# Autodesk Inventor assembly: ASY TZS 1200 Filter column D1200
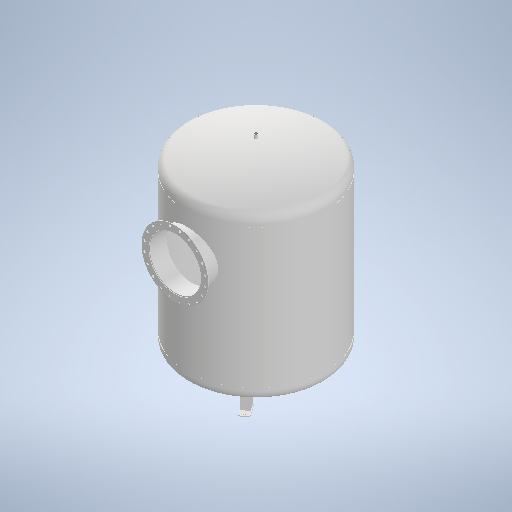
[picture p0: Inventor's stored thumbnail of the model, 512x512]
Saved by Autodesk Inventor 2025 (Build 290162010, 162A)
## iProperties
Created: 2025-02-13
Part Number: ASY TZS 1200 Filter column D1200
Document SubType Name: Assembly
Designer: pokla
Mass: 522904 g
Surface Area: 229381 cm^2
Volume: 66871 cm^3
Density: 7.81959 g/cm^3
Author: pokla
Revision Number: 7
## Documents named in this file (18)
- C:\Users\pokla\Documents\Inventor\TZS-Tazovskiy\ASY TZS 1200 Filter column D1200.iam
- C:\Users\pokla\Documents\Inventor\TZS-Tazovskiy\TZS 1403 accses hatch flange.ipt
- C:\Users\pokla\Documents\Inventor\TZS-Tazovskiy\TZS 1401 DIM Filter column D1200.ipt
- C:\Users\pokla\Documents\Inventor\TZS-Tazovskiy\TZS 14031 accses hatch tube.ipt
- C:\Users\pokla\Documents\Inventor\TZS-Tazovskiy\TZS 1402 SHELL D1200.ipt
- C:\Users\pokla\Documents\Inventor\TZS-Tazovskiy\TZS 1408 dished head.ipt
- C:\Users\pokla\Documents\Inventor\TZS-Tazovskiy\Fitting G1.ipt
- C:\Users\pokla\Documents\Inventor\TZS-Tazovskiy\TZS 1421 charging tube.ipt
- C:\Users\pokla\Documents\Inventor\TZS-Tazovskiy\ASY TZS 1480 Filter legs.iam
- C:\Users\pokla\Documents\Inventor\TZS-Tazovskiy\TZS 1422 charging flange round.ipt
- C:\Users\pokla\Documents\Inventor\TZS-Tazovskiy\sprinkler dummy.ipt
- C:\Users\pokla\Documents\Inventor\TZS-Tazovskiy\ASY TZS 1410 charging hatch.iam
- C:\Users\pokla\Documents\Inventor\TZS-Tazovskiy\TZS 1423 charging flange cup.ipt
- C:\Users\pokla\Documents\Inventor\TZS-Tazovskiy\TZS APN 1430 inner elbow.iam
- C:\Users\pokla\Documents\Inventor\TZS-Tazovskiy\ASY TZS 1440 FDS Top elbow.iam
- C:\Users\pokla\Documents\Inventor\TZS-Tazovskiy\TZS APN 1470 top funnel.iam
- C:\Users\pokla\Documents\Inventor\TZS-Tazovskiy\JIS B 2312 90 Deg Long Elbow Steel 32A x Sch 40.ipt
- C:\Users\pokla\Documents\Inventor\TZS-Tazovskiy\TZS 1491 accses hatch shell.ipt
## Components (58 placed, 17 different names)
1. TZS 1401 DIM Filter column D1200.ipt:1
2. TZS 14031 accses hatch tube.ipt:1 — Rigid:50, Rigid:101
3. TZS 1402 SHELL D1200.ipt:1 — Flush:3, Flush:4, Rigid:99, Rigid:100, Rigid:101, Rigid:102, Rigid:103
4. TZS 1408 dished head.ipt:1 — Rigid:99, Mate:5, Rigid:105
5. TZS 1408 dished head.ipt:2 — Rigid:100, Rigid:104
6. Fitting G1.ipt:1 — Rigid:104
7. APN 1421 charging tube.ipt:1 — Rigid:32
8. TZS 1403 accses hatch flange.ipt:1 — Rotational:4, Rigid:50
9. ASY APN 1480 Filter legs.iam:1 [sub-assembly] — Flush:2, Mate:4, Angle:1
10. APN 1422 charging flange round.ipt:1 — Rigid:32, Rigid:51
11. ASY APN 1410 charging hatch.iam:1 [sub-assembly] — Rotational:4
12. APN 1423 charging flange cup.ipt:1 — Rigid:51
13. ASY APN 1430 inner elbow.iam:1 [sub-assembly] — Rigid:103
14. ASY APN 1440 FDS Top elbow.iam:1 [sub-assembly] — Rigid:97, Rigid:102
15. ASY APN 1470 top funnel.iam:1 [sub-assembly] — Rigid:97
16. JIS B 2312 90 Deg Long Elbow Steel 32A x Sch 40.ipt:1 — Rigid:105
17. ANP 1491 accses hatch shell:1
18. sprinkler dummy.ipt:1
19. sprinkler dummy.ipt:2
20. sprinkler dummy.ipt:3
21. sprinkler dummy.ipt:4
22. sprinkler dummy.ipt:5
23. sprinkler dummy.ipt:6
24. sprinkler dummy.ipt:7
25. sprinkler dummy.ipt:8
26. sprinkler dummy.ipt:9
27. sprinkler dummy.ipt:10
28. sprinkler dummy.ipt:11
29. sprinkler dummy.ipt:12
30. sprinkler dummy.ipt:13
31. sprinkler dummy.ipt:14
32. sprinkler dummy.ipt:15
33. sprinkler dummy.ipt:16
34. sprinkler dummy.ipt:17
35. sprinkler dummy.ipt:18
36. sprinkler dummy.ipt:19
37. sprinkler dummy.ipt:20
38. sprinkler dummy.ipt:21
39. sprinkler dummy.ipt:22
40. sprinkler dummy.ipt:23
41. sprinkler dummy.ipt:24
42. sprinkler dummy.ipt:25
43. sprinkler dummy.ipt:26
44. sprinkler dummy.ipt:27
45. sprinkler dummy.ipt:28
46. sprinkler dummy.ipt:29
47. sprinkler dummy.ipt:30
48. sprinkler dummy.ipt:31
49. sprinkler dummy.ipt:32
50. sprinkler dummy.ipt:33
51. sprinkler dummy.ipt:34
52. sprinkler dummy.ipt:35
53. sprinkler dummy.ipt:36
54. sprinkler dummy.ipt:37
55. sprinkler dummy.ipt:38
56. sprinkler dummy.ipt:39
57. sprinkler dummy.ipt:40
58. sprinkler dummy.ipt:41
## Relationships (18: WeldJoint 11, Flush 3, Mate 2, Angle 1, RevoluteJoint 1)
- Flush:3: TZS 1402 SHELL D1200.ipt:1
- Flush:4: TZS 1402 SHELL D1200.ipt:1
- Flush:2: ASY APN 1480 Filter legs.iam:1
- Rigid:32 [WeldJoint]: APN 1421 charging tube.ipt:1 ↔ APN 1422 charging flange round.ipt:1
- Mate:4: ASY APN 1480 Filter legs.iam:1
- Angle:1 (145 deg): ASY APN 1480 Filter legs.iam:1
- Rotational:4 [RevoluteJoint]: TZS 1403 accses hatch flange.ipt:1 ↔ ASY APN 1410 charging hatch.iam:1
- Rigid:50 [WeldJoint]: TZS 14031 accses hatch tube.ipt:1 ↔ TZS 1403 accses hatch flange.ipt:1
- Rigid:51 [WeldJoint]: APN 1422 charging flange round.ipt:1 ↔ APN 1423 charging flange cup.ipt:1
- Rigid:97 [WeldJoint]: ASY APN 1440 FDS Top elbow.iam:1 ↔ ASY APN 1470 top funnel.iam:1
- Rigid:99 [WeldJoint]: TZS 1402 SHELL D1200.ipt:1 ↔ TZS 1408 dished head.ipt:1
- Rigid:100 [WeldJoint]: TZS 1402 SHELL D1200.ipt:1 ↔ TZS 1408 dished head.ipt:2
- Rigid:101 [WeldJoint]: TZS 14031 accses hatch tube.ipt:1 ↔ TZS 1402 SHELL D1200.ipt:1
- Mate:5 (120 mm): TZS 1408 dished head.ipt:1
- Rigid:102 [WeldJoint] (100 mm): TZS 1402 SHELL D1200.ipt:1 ↔ ASY APN 1440 FDS Top elbow.iam:1
- Rigid:103 [WeldJoint] (100 mm): TZS 1402 SHELL D1200.ipt:1 ↔ ASY APN 1430 inner elbow.iam:1
- Rigid:104 [WeldJoint]: TZS 1408 dished head.ipt:2 ↔ Fitting G1.ipt:1
- Rigid:105 [WeldJoint]: TZS 1408 dished head.ipt:1 ↔ JIS B 2312 90 Deg Long Elbow Steel 32A x Sch 40.ipt:1
